# Autodesk Inventor assembly: Drivetrain Encoder
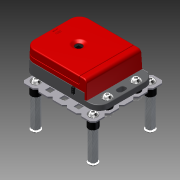
[picture p0: Inventor's stored thumbnail of the model, 180x180]
Saved by Autodesk Inventor 2012 (Build 160160000, 160)
## iProperties
Created: 2011-09-12
Part Number: Drivetrain Encoder
Document SubType Name: Assembly
Designer: Wade
Author: Wade
## Documents named in this file (10)
- C:\Users\Wade\Documents\1103 Robot - CAD Assembly\Drivetrain Encoder.iam
- C:\Users\Wade\Documents\24C VEX CAD Files\Metal Plates\Plate 5x5.ipt
- C:\Users\Wade\Documents\24C VEX CAD Files\Washers & Spacers\Spacer (Thick), 8mm.ipt
- C:\Users\Wade\Documents\24C VEX CAD Files\Standoffs & Couplers\Standoff 1.00''.ipt
- C:\Users\Wade\Documents\24C VEX CAD Files\Motors & Sensors\Optical Shaft (Quadrature) Encoder.iam
- C:\Users\Wade\Documents\24C VEX CAD Files\Washers & Spacers\Spacer (Thin), 4.6mm.ipt
- C:\Users\Wade\Documents\24C VEX CAD Files\Screws & Nuts\Nut 8-32 Nylock.ipt
- C:\Users\Wade\Documents\24C VEX CAD Files\Screws & Nuts\Screw 8-32 x 0.500''-Silver.ipt
- C:\Users\Wade\Documents\1103 Robot - CAD Assembly\Bearing Block.iam
- C:\Users\Wade\Documents\24C VEX CAD Files\Screws & Nuts\Screw 8-32 x 0.250''-Silver.ipt
## Components (25 placed, 9 different names)
1. Plate 5x5:1 — Tangent:1, Tangent:2, Tangent:3, Tangent:4, Tangent:5, Tangent:6, Tangent:7, Tangent:8, Mate:1, Mate:2, Mate:3, Mate:4, Mate:21, Flush:1, Flush:2, Tangent:9, Tangent:10, Tangent:11, Tangent:12, Mate:26, Mate:28, Tangent:13, Tangent:14, Mate:31, Tangent:15, Tangent:16
2. Spacer (Thick), 8mm:1 — Tangent:1, Tangent:2, Mate:1, Mate:7, Mate:12
3. Spacer (Thick), 8mm:2 — Tangent:3, Tangent:4, Mate:3, Mate:6, Mate:9
4. Spacer (Thick), 8mm:3 — Tangent:7, Tangent:8, Mate:2, Mate:8, Mate:11
5. Spacer (Thick), 8mm:4 — Tangent:5, Tangent:6, Mate:4, Mate:5, Mate:10
6. Standoff 1.00'':1 — Mate:5, Mate:10, Mate:34, Mate:39
7. Standoff 1.00'':2 — Mate:8, Mate:11, Mate:35, Mate:36
8. Standoff 1.00'':3 — Mate:7, Mate:12, Mate:32, Mate:37
9. Standoff 1.00'':4 — Mate:6, Mate:9, Mate:33, Mate:38
10. Screw 8-32 x 0.500''-Silver:1
11. Screw 8-32 x 0.500''-Silver:2
12. Screw 8-32 x 0.500''-Silver:3
13. Screw 8-32 x 0.500''-Silver:4
14. Optical Shaft (Quadrature) Encoder:1 [sub-assembly] — Mate:21, Mate:30, Tangent:16
15. Spacer (Thin), 4.6mm:1 — Flush:1, Tangent:9, Tangent:10
16. Spacer (Thin), 4.6mm:2 — Flush:2, Tangent:11, Tangent:12
17. Screw 8-32 x 0.500''-Silver:5
18. Screw 8-32 x 0.500''-Silver:6
19. Nut 8-32 Nylock:1 — Mate:26
20. Nut 8-32 Nylock:2 — Mate:28
21. Bearing Block:1 [sub-assembly] — Mate:30, Tangent:13, Tangent:14, Mate:31, Tangent:15
22. Screw 8-32 x 0.250''-Silver:1 — Mate:35, Mate:36
23. Screw 8-32 x 0.250''-Silver:2 — Mate:34, Mate:39
24. Screw 8-32 x 0.250''-Silver:3 — Mate:33, Mate:38
25. Screw 8-32 x 0.250''-Silver:4 — Mate:32, Mate:37
## Relationships (57: Mate 39, Tangent 16, Flush 2)
- Tangent:1 (0.1905 mm): Plate 5x5:1 ↔ Spacer (Thick), 8mm:1
- Tangent:2 (0.1905 mm): Plate 5x5:1 ↔ Spacer (Thick), 8mm:1
- Tangent:3 (0.1905 mm): Plate 5x5:1 ↔ Spacer (Thick), 8mm:2
- Tangent:4 (0.1905 mm): Plate 5x5:1 ↔ Spacer (Thick), 8mm:2
- Tangent:5 (0.1905 mm): Plate 5x5:1 ↔ Spacer (Thick), 8mm:4
- Tangent:6 (0.1905 mm): Plate 5x5:1 ↔ Spacer (Thick), 8mm:4
- Tangent:7 (0.1905 mm): Plate 5x5:1 ↔ Spacer (Thick), 8mm:3
- Tangent:8 (0.1905 mm): Plate 5x5:1 ↔ Spacer (Thick), 8mm:3
- Mate:1: Plate 5x5:1 ↔ Spacer (Thick), 8mm:1
- Mate:2: Plate 5x5:1 ↔ Spacer (Thick), 8mm:3
- Mate:3: Plate 5x5:1 ↔ Spacer (Thick), 8mm:2
- Mate:4: Plate 5x5:1 ↔ Spacer (Thick), 8mm:4
- Mate:5: Spacer (Thick), 8mm:4 ↔ Standoff 1.00'':1
- Mate:6: Spacer (Thick), 8mm:2 ↔ Standoff 1.00'':4
- Mate:7: Spacer (Thick), 8mm:1 ↔ Standoff 1.00'':3
- Mate:8: Spacer (Thick), 8mm:3 ↔ Standoff 1.00'':2
- Mate:9: Spacer (Thick), 8mm:2 ↔ Standoff 1.00'':4
- Mate:10: Spacer (Thick), 8mm:4 ↔ Standoff 1.00'':1
- Mate:11: Spacer (Thick), 8mm:3 ↔ Standoff 1.00'':2
- Mate:12: Spacer (Thick), 8mm:1 ↔ Standoff 1.00'':3
- [Mate]: Spacer (Thick), 8mm:2 ↔ Screw 8-32 x 0.500''-Silver:1
- [Mate]: Spacer (Thick), 8mm:4 ↔ Screw 8-32 x 0.500''-Silver:2
- [Mate]: Spacer (Thick), 8mm:1 ↔ Screw 8-32 x 0.500''-Silver:3
- [Mate]: Spacer (Thick), 8mm:3 ↔ Screw 8-32 x 0.500''-Silver:4
- [Mate]: Plate 5x5:1 ↔ Screw 8-32 x 0.500''-Silver:1
- [Mate]: Plate 5x5:1 ↔ Screw 8-32 x 0.500''-Silver:3
- [Mate]: Plate 5x5:1 ↔ Screw 8-32 x 0.500''-Silver:2
- [Mate]: Plate 5x5:1 ↔ Screw 8-32 x 0.500''-Silver:4
- Mate:21 (2.54 mm): Plate 5x5:1 ↔ Optical Shaft (Quadrature) Encoder:1
- Flush:1: Plate 5x5:1 ↔ Spacer (Thin), 4.6mm:1
- Flush:2: Plate 5x5:1 ↔ Spacer (Thin), 4.6mm:2
- Tangent:9 (0.1905 mm): Plate 5x5:1 ↔ Spacer (Thin), 4.6mm:1
- Tangent:10 (0.1905 mm): Plate 5x5:1 ↔ Spacer (Thin), 4.6mm:1
- Tangent:11 (0.1905 mm): Plate 5x5:1 ↔ Spacer (Thin), 4.6mm:2
- Tangent:12 (0.1905 mm): Plate 5x5:1 ↔ Spacer (Thin), 4.6mm:2
- [Mate]: Spacer (Thin), 4.6mm:1 ↔ Screw 8-32 x 0.500''-Silver:5
- [Mate]: Spacer (Thin), 4.6mm:2 ↔ Screw 8-32 x 0.500''-Silver:6
- [Mate]: Optical Shaft (Quadrature) Encoder:1 ↔ Screw 8-32 x 0.500''-Silver:5
- [Mate]: Optical Shaft (Quadrature) Encoder:1 ↔ Screw 8-32 x 0.500''-Silver:6
- Mate:26: Plate 5x5:1 ↔ Nut 8-32 Nylock:1
- [Mate]: Screw 8-32 x 0.500''-Silver:5 ↔ Nut 8-32 Nylock:1
- Mate:28: Plate 5x5:1 ↔ Nut 8-32 Nylock:2
- [Mate]: Screw 8-32 x 0.500''-Silver:6 ↔ Nut 8-32 Nylock:2
- Mate:30: Optical Shaft (Quadrature) Encoder:1 ↔ Bearing Block:1
- Tangent:13 (0.1905 mm): Plate 5x5:1 ↔ Bearing Block:1
- Tangent:14 (0.1905 mm): Plate 5x5:1 ↔ Bearing Block:1
- Mate:31: Plate 5x5:1 ↔ Bearing Block:1
- Tangent:15 (0.1905 mm): Plate 5x5:1 ↔ Bearing Block:1
- Tangent:16 (-1.524 mm): Plate 5x5:1 ↔ Optical Shaft (Quadrature) Encoder:1
- Mate:32 (1.1684 mm): Standoff 1.00'':3 ↔ Screw 8-32 x 0.250''-Silver:4
- Mate:33 (1.1684 mm): Standoff 1.00'':4 ↔ Screw 8-32 x 0.250''-Silver:3
- Mate:34 (1.1684 mm): Standoff 1.00'':1 ↔ Screw 8-32 x 0.250''-Silver:2
- Mate:35 (1.1684 mm): Standoff 1.00'':2 ↔ Screw 8-32 x 0.250''-Silver:1
- Mate:36: Standoff 1.00'':2 ↔ Screw 8-32 x 0.250''-Silver:1
- Mate:37: Standoff 1.00'':3 ↔ Screw 8-32 x 0.250''-Silver:4
- Mate:38: Standoff 1.00'':4 ↔ Screw 8-32 x 0.250''-Silver:3
- Mate:39: Standoff 1.00'':1 ↔ Screw 8-32 x 0.250''-Silver:2
